# Autodesk Inventor assembly: Slew Bearing v2 v18
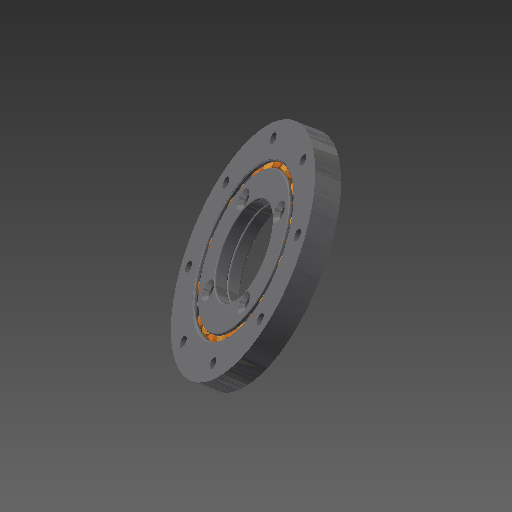
[picture p0: Inventor's stored thumbnail of the model, 512x512]
Saved by Autodesk Inventor 2020 (Build 240168000, 168)
## iProperties
Created: 2020-05-22
Part Number: Slew Bearing v2 v18
Document SubType Name: Assembly
Designer: Administrator
Title: Slew Bearing v2 v18 v7
Author: Administrator
## Documents named in this file (5)
- D:\github_gedeeld\BeerMinder\3D-model\bearings\slewbearing\Slew Bearing v2 v18.iam
- D:\github_gedeeld\BeerMinder\3D-model\bearings\slewbearing\Rolls A.ipt
- D:\github_gedeeld\BeerMinder\3D-model\bearings\slewbearing\Rolls B.ipt
- D:\github_gedeeld\BeerMinder\3D-model\bearings\slewbearing\Race Outer.ipt
- D:\github_gedeeld\BeerMinder\3D-model\bearings\slewbearing\Race Inner.iam
## Components (4 placed, 4 different names)
1. Rolls A:1 — Mate:1, Mate:5, Angle:1
2. Rolls B:1 — Mate:2, Mate:4, Angle:1
3. Race Outer:1 — Mate:1, Mate:2, Flush:4, Mate:4, Mate:5, Mate:6
4. Race Inner:1 [sub-assembly] — Flush:4, Mate:6
## Relationships (7: Mate 5, Flush 1, Angle 1)
- Mate:1: Rolls A:1 ↔ Race Outer:1
- Mate:2: Rolls B:1 ↔ Race Outer:1
- Flush:4: Race Outer:1 ↔ Race Inner:1
- Mate:4: Rolls B:1 ↔ Race Outer:1
- Mate:5: Rolls A:1 ↔ Race Outer:1
- Mate:6: Race Outer:1 ↔ Race Inner:1
- Angle:1 (28.2 deg): Rolls A:1 ↔ Rolls B:1
